# Autodesk Inventor assembly: 000.005.006 - Захват СБ
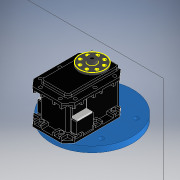
[picture p0: Inventor's stored thumbnail of the model, 180x180]
Saved by Autodesk Inventor 2022 (Build 260153000, 153)
## iProperties
Created: 2022-12-20
Part Number: 000.005.006 - Захват СБ
Document SubType Name: Assembly
Designer: Ivan Petrov
Author: Ivan Petrov
## Documents named in this file (3)
- C:\Users\Ivan Petrov\Documents\GitHub\OmniBot\design\000.005.006 - Захват СБ.iam
- C:\Users\Ivan Petrov\Documents\GitHub\OmniBot\design\000.005.006.001 - Основание.ipt
- C:\Users\Ivan Petrov\Documents\GitHub\OmniBot\design\standart_components\dynamixels\mx-28\MX-28.iam
## Components (2 placed, 2 different names)
1. 000.005.006.001 - Основание:1 — Совмещение:1, Совмещение:2
2. MX-28:1 [sub-assembly] — Совмещение:1, Совмещение:2, Угол:1
## Relationships (3: Mate 2, Angle 1)
- Совмещение:1 [Mate]: 000.005.006.001 - Основание:1 ↔ MX-28:1
- Совмещение:2 [Mate]: 000.005.006.001 - Основание:1 ↔ MX-28:1
- Угол:1 [Angle] (0 deg): MX-28:1
